# Autodesk Inventor assembly: 足首_独立ピッチ_1
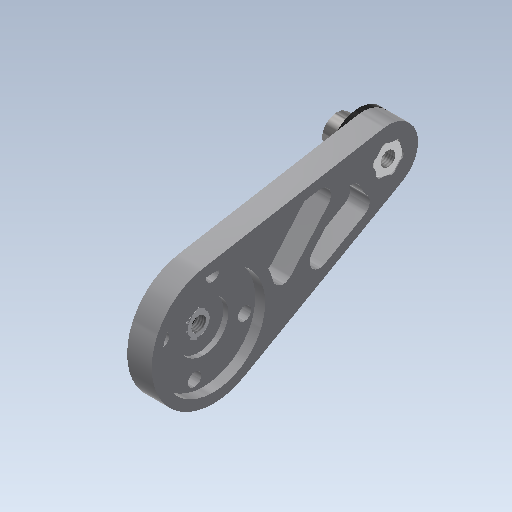
[picture p0: Inventor's stored thumbnail of the model, 512x512]
Saved by Autodesk Inventor 2020.4 (Build 244396000, 396)
## iProperties
Created: 2016-05-04
Part Number: 足首_独立ピッチ_1
Document SubType Name: Assembly
Designer: hiroaki
Mass: 8.82988 g
Surface Area: 48.3734 cm^2
Volume: 3.02944 cm^3
Density: 2.9147 g/cm^3
Author: hiroaki
## Documents named in this file (6)
- C:\Users\Masato\Documents\Inventor\CIT Brains_Inventor\OpenPlatform_ver3_0\下半身\足首\足首_独立ピッチ_1.iam
- C:\Users\Masato\Documents\Inventor\CIT Brains_Inventor\OpenPlatform_ver3_0\下半身\足首\足首_独立ピッチ_1_1.ipt
- C:\Users\Masato\Documents\Inventor\CIT Brains_Inventor\OpenPlatform_ver3_0\Ready_Made\S3-07-3W.ipt
- C:\Users\Masato\Documents\Inventor\CIT Brains_Inventor\OpenPlatform_ver3_0\Ready_Made\UUW-0312-10BH.ipt
- C:\Users\Masato\Documents\Inventor\CIT Brains_Inventor\OpenPlatform_ver3_0\Ready_Made\CU-304.5H.ipt
- C:\Users\Masato\Documents\Inventor\CIT Brains_Inventor\OpenPlatform_ver3_0\Ready_Made\SF319.ipt
## Components (7 placed, 5 different names)
1. 足首_独立ピッチ_1_1:1 — 挿入:6, 挿入:7, メイト:1, 挿入:14, 挿入:15
2. S3-07-3W:1 — 挿入:6, メイト:1
3. UUW-0312-10BH:1 — 挿入:7
4. UUW-0312-10BH:2 — 挿入:15
5. CU-304.5H:1
6. CU-304.5H:2
7. SF319:1 — 挿入:14
## Relationships (5: Insert 4, Mate 1)
- 挿入:6 [Insert]: 足首_独立ピッチ_1_1:1 ↔ S3-07-3W:1
- 挿入:7 [Insert]: 足首_独立ピッチ_1_1:1 ↔ UUW-0312-10BH:1
- メイト:1 [Mate] (0.01 mm): 足首_独立ピッチ_1_1:1 ↔ S3-07-3W:1
- 挿入:14 [Insert]: 足首_独立ピッチ_1_1:1 ↔ SF319:1
- 挿入:15 [Insert]: 足首_独立ピッチ_1_1:1 ↔ UUW-0312-10BH:2
